# Autodesk Inventor assembly: 부피 구하기3
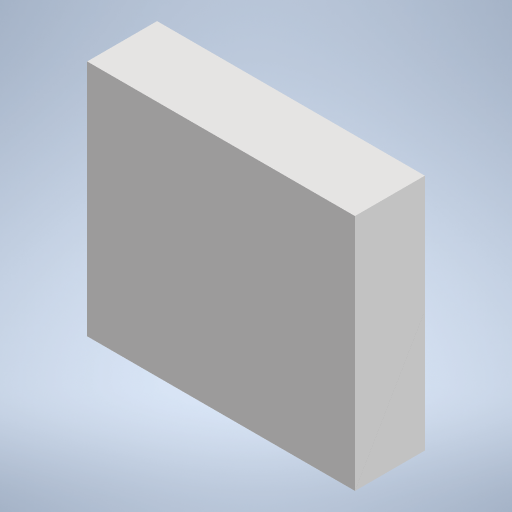
[picture p0: Inventor's stored thumbnail of the model, 512x512]
Saved by Autodesk Inventor 2024 (Build 280153000, 153)
## iProperties
Created: 2023-06-26
Part Number: 부피 구하기3
Document SubType Name: Assembly
Designer: jsw
Author: jsw
## Documents named in this file (3)
- C:\승원\co-op\OV-PAM\OV-PAM_modeling\부피 구하기3.iam
- C:\승원\co-op\OV-PAM\OV-PAM_modeling\부피 구하기3.ipt
- C:\승원\co-op\OV-PAM\OV-PAM_modeling\부피 구하기4.ipt
## Components (2 placed, 2 different names)
1. 부피 구하기3:1 — 메이트:1, 메이트:2
2. 부피 구하기4:1 — 메이트:1, 메이트:2
## Relationships (2: Mate 2)
- 메이트:1 [Mate]: 부피 구하기3:1 ↔ 부피 구하기4:1
- 메이트:2 [Mate]: 부피 구하기3:1 ↔ 부피 구하기4:1
